# Autodesk Inventor assembly: krancowka_uchwyt_alternatywa_2
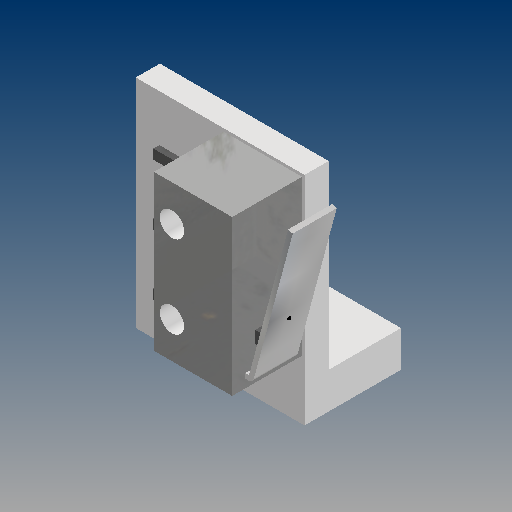
[picture p0: Inventor's stored thumbnail of the model, 512x512]
Saved by Autodesk Inventor 2021 (Build 250183000, 183)
## iProperties
Created: 2022-09-08
Part Number: krancowka_uchwyt_alternatywa_2
Document SubType Name: Assembly
Designer: agnpi
Author: agnpi
## Documents named in this file (3)
- E:\Users\agnpi\Desktop\lekcje\SEMESTR VI\inzynierka\Uchwyt - robot\krancowka_uchwyt_alternatywa_2_.iam
- E:\Users\agnpi\Desktop\lekcje\SEMESTR VI\inzynierka\Chwytak podejscie 2\uchwyt_krancowka_alternatywa_2.ipt
- E:\Users\agnpi\Desktop\lekcje\SEMESTR VI\inzynierka\Chwytak podejscie 2\krancowka.ipt
## Components (2 placed, 2 different names)
1. uchwyt_krancowka_alternatywa_2:1 — Mate:1, Angle:1, Angle:2
2. krancowka:1 — Mate:1, Angle:1, Angle:2
## Relationships (3: Angle 2, Mate 1)
- Mate:1: uchwyt_krancowka_alternatywa_2:1 ↔ krancowka:1
- Angle:1 (180 deg): uchwyt_krancowka_alternatywa_2:1 ↔ krancowka:1
- Angle:2 (180 deg): uchwyt_krancowka_alternatywa_2:1 ↔ krancowka:1
